# Autodesk Inventor assembly: 211-01
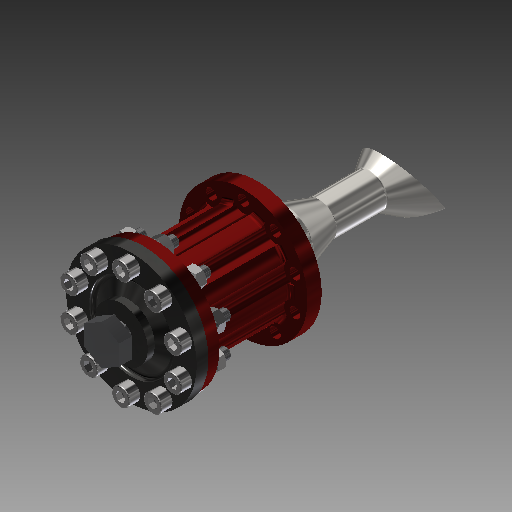
[picture p0: Inventor's stored thumbnail of the model, 512x512]
Saved by Autodesk Inventor 2019 (Build 230136000, 136)
## iProperties
Company: Autodesk Inc.
Created: 2017-03-15
Part Number: 211-01
Document SubType Name: Assembly
Designer: Autodesk Inc.
Mass: 372.996 g
Surface Area: 560.921 cm^2
Volume: 66.0055 cm^3
Density: 5.65098 g/cm^3
Author: Inventor
## Documents named in this file (6)
- C:\TEMP\Jet Engine Model\Workspace\Front Compression Fan\Combustion Chamber.iam
- C:\TEMP\Jet Engine Model\Workspace\Front Compression Fan\Combustion Casing.ipt
- C:\TEMP\Jet Engine Model\Workspace\Front Compression Fan\Combustion Chamber.ipt
- C:\TEMP\Jet Engine Model\Workspace\Front Compression Fan\Combustion Cap.ipt
- C:\TEMP\Jet Engine Model\Workspace\Front Compression Fan\Fuel Port Cap.ipt
- C:\TEMP\Jet Engine Model\Workspace\Design Accelerator\Bolted Connection2.iam
## Components (14 placed, 5 different names)
1. Combustion Casing:1 — Insert:2, Insert:3, Mate:5, Flush:1, Mate:6
2. Combustion Chamber:1 — Mate:2, Flush:2
3. Combustion Cap:1 — Insert:2, Insert:3, Mate:1, Insert:4, Mate:3, Mate:4
4. Fuel Port Cap:1 — Mate:1, Insert:4, Mate:2
5. Bolted Connection:1 [sub-assembly] — Mate:3, Mate:4
6. Bolted Connection:2 [sub-assembly]
7. Bolted Connection:3 [sub-assembly]
8. Bolted Connection:4 [sub-assembly]
9. Bolted Connection:5 [sub-assembly]
10. Bolted Connection:6 [sub-assembly]
11. Bolted Connection:7 [sub-assembly]
12. Bolted Connection:8 [sub-assembly]
13. Bolted Connection:9 [sub-assembly]
14. Bolted Connection:10 [sub-assembly]
## Component patterns: (10 elements, first: Bolted Connection:1)
## Relationships (12: Mate 6, Insert 4, Flush 2)
- [Insert] (-21.89 mm): Combustion Casing:1 ↔ Combustion Chamber:1
- Insert:2: Combustion Casing:1 ↔ Combustion Cap:1
- Insert:3: Combustion Casing:1 ↔ Combustion Cap:1
- Mate:1: Combustion Cap:1 ↔ Fuel Port Cap:1
- Insert:4: Combustion Cap:1 ↔ Fuel Port Cap:1
- Mate:2: Combustion Chamber:1 ↔ Fuel Port Cap:1
- Mate:3: Combustion Cap:1 ↔ Bolted Connection:1
- Mate:4: Combustion Cap:1 ↔ Bolted Connection:1
- Mate:5: Combustion Casing:1
- Flush:1: Combustion Casing:1
- Mate:6: Combustion Casing:1
- Flush:2: Combustion Chamber:1
